# Autodesk Inventor assembly: Motor_Panel
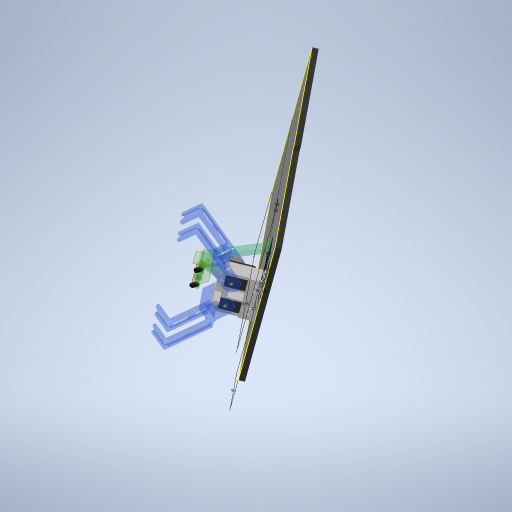
[picture p0: Inventor's stored thumbnail of the model, 512x512]
Saved by Autodesk Inventor 2023 (Build 270158000, 158)
## iProperties
Created: 2019-09-17
Part Number: Motor_Panel
Document SubType Name: Assembly
Designer: Knowblesse
Author: Knowblesse
## Documents named in this file (10)
- C:\VCF\Lobster\Apparatus\Robot\Motor_Panel.iam
- C:\VCF\Lobster\Apparatus\Robot\Motor.ipt
- C:\VCF\Lobster\Apparatus\Robot\Motor_disk.ipt
- C:\VCF\Lobster\Apparatus\Robot\MotorBracket.ipt
- C:\VCF\Lobster\Apparatus\Arena\Board.ipt
- C:\VCF\Lobster\Apparatus\Lick\LickSensor.ipt
- C:\VCF\Lobster\Apparatus\Lick\LickLight.ipt
- C:\VCF\Lobster\Apparatus\Robot\Claw.ipt
- C:\VCF\Lobster\Apparatus\Lick\Lick.iam
- C:\VCF\Lobster\Apparatus\Robot\Claw_MIR.ipt
## Components (12 placed, 9 different names)
1. Motor:1 — 회전:1, 강체:1
2. Motor:2 — 회전:2, 강체:2
3. Motor_disk:1 — 회전:2, 회전:4, 강체:10
4. Motor_disk:2 — 회전:1
5. MotorBracket:1 — 강체:1, 강체:2, 강체:15, 각도:2
6. Board:1 — 강체:15, 강체:16
7. LickSensor:1 — 강체:8, 강체:20
8. LickSensor:2 — 강체:19
9. LickLight:1 — 강체:8
10. Claw:1 — 회전:4, 강체:10, 각도:2
11. Claw_MIR:1
12. Lick:1 [sub-assembly] — 강체:16, 강체:19, 강체:20
## Relationships (12: WeldJoint 8, RevoluteJoint 3, Angle 1)
- 회전:1 [RevoluteJoint]: Motor:1 ↔ Motor_disk:2
- 회전:2 [RevoluteJoint]: Motor:2 ↔ Motor_disk:1
- 강체:1 [WeldJoint]: Motor:1 ↔ MotorBracket:1
- 강체:2 [WeldJoint]: Motor:2 ↔ MotorBracket:1
- 강체:8 [WeldJoint]: LickSensor:1 ↔ LickLight:1
- 회전:4 [RevoluteJoint]: Motor_disk:1 ↔ Claw:1
- 강체:10 [WeldJoint]: Motor_disk:1 ↔ Claw:1
- 강체:15 [WeldJoint]: MotorBracket:1 ↔ Board:1
- 강체:16 [WeldJoint]: Board:1 ↔ Lick:1
- 각도:2 [Angle] (0 deg): MotorBracket:1 ↔ Claw:1
- 강체:19 [WeldJoint]: LickSensor:2 ↔ Lick:1
- 강체:20 [WeldJoint]: LickSensor:1 ↔ Lick:1
